# Autodesk Inventor assembly: NEW ASSEM
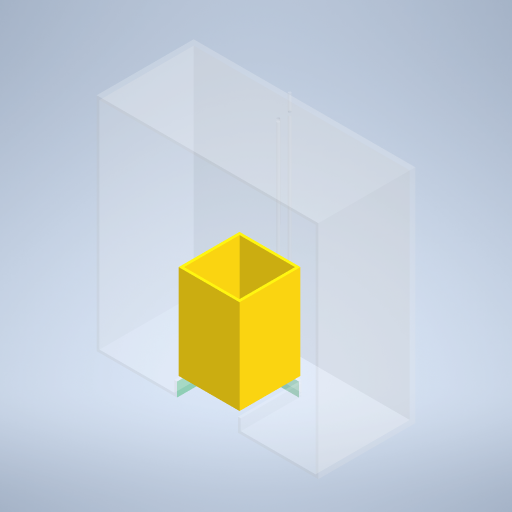
[picture p0: Inventor's stored thumbnail of the model, 512x512]
Saved by Autodesk Inventor 2024 (Build 280153000, 153)
## iProperties
Created: 2023-06-03
Part Number: NEW ASSEM
Document SubType Name: Assembly
Designer: hithi
Author: hithi
## Documents named in this file (3)
- C:\Users\hithi\OneDrive\Desktop\NEW ASSEM.iam
- C:\Users\hithi\OneDrive\Desktop\NEW1.ipt
- C:\Users\hithi\Downloads\EE1.ipt
## Components (2 placed, 2 different names)
1. NEW1:1 — Mate:1, Mate:2, Mate:3
2. EE1:1 — Mate:1, Mate:2, Mate:3
## Relationships (3: Mate 3)
- Mate:1: NEW1:1 ↔ EE1:1
- Mate:2: NEW1:1 ↔ EE1:1
- Mate:3: NEW1:1 ↔ EE1:1
